# Autodesk Inventor assembly: Marco_apm_001-1
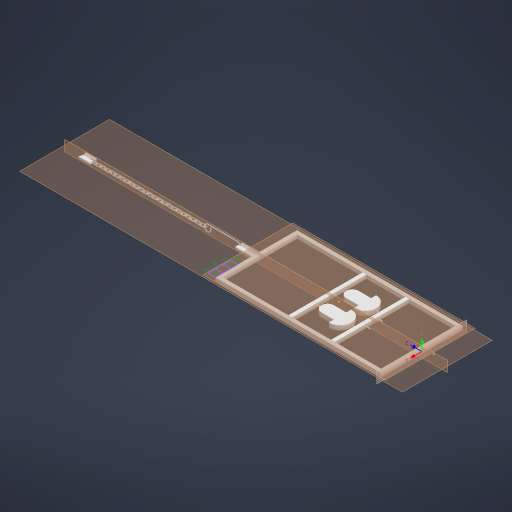
[picture p0: Inventor's stored thumbnail of the model, 512x512]
Saved by Autodesk Inventor 2024 (Build 280153000, 153)
## iProperties
Created: 2023-05-17
Part Number: Marco_apm_001-1
Document SubType Name: Assembly
Designer: javie
Author: javie
## Documents named in this file (8)
- C:\Users\javie\Downloads\Piezas CMR\Marco_APM_001\Marco_apm_001-1.iam
- C:\Users\javie\Downloads\Piezas CMR\Marco_Conveyor_Aereo.iam
- C:\Users\javie\Downloads\Piezas CMR\Marcos_solids\Topes_apm_002-2.ipt
- C:\Users\javie\Downloads\Piezas CMR\Marcos_solids\S_horizontal.ipt
- C:\Users\javie\Downloads\Piezas CMR\Marco_APM_002\Piezas\APM_002-5.ipt
- C:\Users\javie\Downloads\Piezas CMR\Marcos_solids\Topes_apm_2.ipt
- C:\Users\javie\Downloads\Piezas CMR\Marco_APM_001\Partes\APM_001-1.ipt
- C:\Users\javie\Downloads\Piezas CMR\Marcos_solids\000.ipt
## Components (11 placed, 7 different names)
1. Marco_Conveyor_Aereo:1 [sub-assembly] — Nivelación:5, Nivelación:6
2. Topes_apm_002-2:1 — Insertar:3
3. S_horizontal:1 — Insertar:3, Nivelación:3, Nivelación:4
4. APM_002-5:1 — Insertar:4
5. APM_002-5:2 — Insertar:5
6. Topes_apm_2:1 — Nivelación:3, Nivelación:4, Insertar:4, Insertar:5, Cilíndrica:1, Cilíndrica:2
7. S_horizontal:2 — Insertar:6, Insertar:7
8. APM_001-1:1 — Cilíndrica:1
9. APM_001-1:2 — Cilíndrica:2
10. Topes_apm_2:2 — Insertar:6, Insertar:7
11. 000:1 — Nivelación:5, Nivelación:6
## Relationships (11: Insert 5, Flush 4, CylindricalJoint 2)
- Insertar:3: Topes_apm_002-2:1 ↔ S_horizontal:1
- Nivelación:3 [Flush]: S_horizontal:1 ↔ Topes_apm_2:1
- Nivelación:4 [Flush]: S_horizontal:1 ↔ Topes_apm_2:1
- Insertar:4: APM_002-5:1 ↔ Topes_apm_2:1
- Insertar:5: APM_002-5:2 ↔ Topes_apm_2:1
- Cilíndrica:1 [CylindricalJoint]: Topes_apm_2:1 ↔ APM_001-1:1
- Cilíndrica:2 [CylindricalJoint]: Topes_apm_2:1 ↔ APM_001-1:2
- Insertar:6: S_horizontal:2 ↔ Topes_apm_2:2
- Insertar:7: S_horizontal:2 ↔ Topes_apm_2:2
- Nivelación:5 [Flush]: Marco_Conveyor_Aereo:1 ↔ 000:1
- Nivelación:6 [Flush]: Marco_Conveyor_Aereo:1 ↔ 000:1
